# Autodesk Inventor assembly: Electrode_assembly_v6
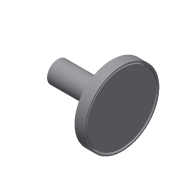
[picture p0: Inventor's stored thumbnail of the model, 180x180]
Saved by Autodesk Inventor 2013 (Build 170138000, 138)
## iProperties
Created: 2012-06-12
Part Number: Electrode_assembly_v6
Document SubType Name: Assembly
Designer: Breckenridge2 User
Author: Breckenridge2 User
## Documents named in this file (4)
- D:\Work_Suranga\3d_drawing_of_the_chamber\Educational_version\Electrode_assembly_v6.iam
- D:\Work_Suranga\3d_drawing_of_the_chamber\Electrode_v_1.ipt
- D:\Work_Suranga\3d_drawing_of_the_chamber\Teflon_spacer_v_1.ipt
- D:\Work_Suranga\3d_drawing_of_the_chamber\Educational_version\Assembly1.iam
## Components (3 placed, 3 different names)
1. Electrode_v_1:1 — Insert:2
2. Teflon_spacer_v_1:1 — Insert:1, Insert:2
3. Assembly1:1 [sub-assembly] — Insert:1
## Relationships (2: Insert 2)
- Insert:1: Teflon_spacer_v_1:1 ↔ Assembly1:1
- Insert:2: Electrode_v_1:1 ↔ Teflon_spacer_v_1:1
